# Autodesk Inventor assembly: Traffic signal
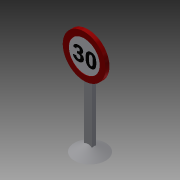
[picture p0: Inventor's stored thumbnail of the model, 180x180]
Saved by Autodesk Inventor 2014 (Build 180170000, 170)
## iProperties
Created: 2017-08-29
Part Number: Traffic signal
Document SubType Name: Assembly
Designer: resaj
Author: resaj
## Documents named in this file (6)
- C:\Users\resaj\GitHub\my-3D-printing-designs\Traffic sign\Traffic sign.iam
- C:\Users\resaj\GitHub\my-3D-printing-designs\Traffic sign\Rim.ipt
- C:\Users\resaj\GitHub\my-3D-printing-designs\Traffic sign\Inside.ipt
- C:\Users\resaj\GitHub\my-3D-printing-designs\Traffic sign\30.ipt
- C:\Users\resaj\GitHub\my-3D-printing-designs\Traffic sign\Pole.ipt
- C:\Users\resaj\GitHub\my-3D-printing-designs\Traffic sign\Base.ipt
## Components (5 placed, 5 different names)
1. Rim:1 — Mate:1, Flush:1
2. Inside:1 — Mate:1, Flush:1, Mate:2, Mate:3, Mate:4, Mate:5, Mate:7, Angle:2
3. 30:1 — Mate:2, Mate:3
4. Pole:1 — Mate:4, Mate:5, Mate:6, Angle:1, Flush:2, Mate:9, Angle:3, Mate:10, Angle:4
5. Base:1 — Flush:2, Mate:11, Angle:5, Mate:12, Angle:6
## Relationships (22: Mate 14, Angle 6, Flush 2)
- Mate:1: Rim:1 ↔ Inside:1
- Flush:1: Rim:1 ↔ Inside:1
- Mate:2: Inside:1 ↔ 30:1
- Mate:3: Inside:1 ↔ 30:1
- Mate:4: Inside:1 ↔ Pole:1
- Mate:5: Inside:1 ↔ Pole:1
- Mate:6: Pole:1
- Angle:1 (0 deg): Pole:1
- Mate:7: Inside:1
- Angle:2 (0 deg): Inside:1
- Mate:8
- Flush:2: Pole:1 ↔ Base:1
- Mate:9: Pole:1
- Angle:3 (0 deg): Pole:1
- Mate:10: Pole:1
- Angle:4 (0 deg): Pole:1
- Mate:11: Base:1
- Angle:5 (0 deg): Base:1
- Mate:12: Base:1
- Angle:6 (0 deg): Base:1
- Mate:13
- Mate:14
